# Autodesk Inventor assembly: 412
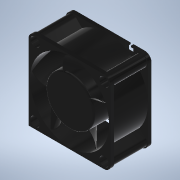
[picture p0: Inventor's stored thumbnail of the model, 180x180]
Saved by Autodesk Inventor 2020 (Build 240168000, 168)
## iProperties
Category: FIRSTChoice
Company: Autodesk Inc.
Part Number: 412
Document SubType Name: Assembly
Created: 2019-11-30
Designer: Autodesk Inc.
Description: Comapct fan - mini 12V DC
Catalog Web Link: https://www.ebmpapst.us/en/products/compact_fans/axial_compact_fans/axial_compact_fans_detail.php?pID=53733
Vendor: ebmpapst
Control State: 0
Master: False
Checked Out: False
Shininess: 64.0
Length Units: 11272
Angle Units: 11279
Time Units: 11290
Mass Units: 11286
Length Display Precision: 3
Angle Display Precision: 2
Compacted: True
Density: 0.0
Volumn: 0.0
Area: 0.0
PropertySet Name: Model Information
Author: Autodesk Inc.
## Documents named in this file (3)
- D:\FIRST 2020\FRC 2020\FRC FIRSTChoice 2020\Inventor\412.iam
- D:\FIRST 2020\FRC 2020\FRC FIRSTChoice 2020\Inventor\Parts\fan body.ipt
- D:\FIRST 2020\FRC 2020\FRC FIRSTChoice 2020\Inventor\Parts\fan blade.ipt
## Components (2 placed, 2 different names)
1. fan body:1 — Flush:1, Mate:1
2. fan blade:1 — Flush:1, Mate:1
## Relationships (2: Flush 1, Mate 1)
- Flush:1: fan body:1 ↔ fan blade:1
- Mate:1: fan body:1 ↔ fan blade:1
